# Autodesk Inventor assembly: Frame with winch
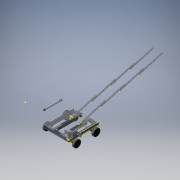
[picture p0: Inventor's stored thumbnail of the model, 180x180]
Saved by Autodesk Inventor 2016 (Build 200138000, 138)
## iProperties
Created: 2015-12-09
Part Number: Frame with winch
Document SubType Name: Assembly
Designer: Julia
Author: Julia
## Documents named in this file (11)
- C:\Users\Julia\Documents\GitHub\RobotuxCAD\FTC CAD Parts\Frame with winch.iam
- C:\Users\Julia\Documents\GitHub\RobotuxCAD\FTC CAD Parts\Frame With Wheels.iam
- C:\Users\Julia\Documents\GitHub\RobotuxCAD\FTC CAD Parts\Tetrix_Kit_FTC\tetrix_739079_collar_2012.ipt
- C:\Users\Julia\Documents\GitHub\RobotuxCAD\FTC CAD Parts\Andy Mark\am-2964NeveRest.ipt
- C:\Users\Julia\Documents\GitHub\RobotuxCAD\FTC CAD Parts\Tetrix_Kit_FTC\tetrix_739089_2012.ipt
- C:\Users\Julia\Documents\GitHub\RobotuxCAD\FTC CAD Parts\Tetrix_Kit_FTC\tetrix_739086_2012.ipt
- C:\Users\Julia\Documents\GitHub\RobotuxCAD\FTC CAD Parts\Tetrix_Kit_FTC\tetrix_739028_2012.ipt
- C:\Users\Julia\Documents\GitHub\RobotuxCAD\FTC CAD Parts\support.ipt
- C:\Users\Julia\Documents\GitHub\RobotuxCAD\FTC CAD Parts\Tetrix_Kit_FTC\tetrix_739172_2012.ipt
- C:\Users\Julia\Documents\GitHub\RobotuxCAD\FTC CAD Parts\tube_clamp_2012.ipt
- C:\Users\Julia\Documents\GitHub\RobotuxCAD\FTC CAD Parts\winch spool.ipt
## Components (13 placed, 10 different names)
1. tetrix_739079_collar_2012:1 — Mate:6, Mate:8, Mate:9
2. am-2964NeveRest:1 — Mate:4, Mate:5, Angle:1, Mate:6, Mate:7
3. tetrix_739089_2012:1 — Mate:1, Mate:2, Mate:3, Mate:4, Mate:5
4. tetrix_739086_2012:1 — Mate:7, Mate:8, Mate:9
5. Frame With Wheels:1 [sub-assembly] — Mate:1, Mate:2, Mate:3, Angle:1, Flush:1, Flush:2, Mate:10, Mate:11
6. tetrix_739028_2012:1 — Mate:12, Mate:13, Mate:14, Mate:15, Mate:16
7. support:1 — Flush:1, Flush:2, Mate:10, Mate:11, Mate:12, Mate:13
8. tetrix_739172_2012:1 — Mate:14, Mate:15, Mate:16
9. tetrix_739172_2012:2 — Mate:17, Mate:19, Mate:22, Mate:23
10. tetrix_739172_2012:3 — Mate:18, Mate:20, Mate:21, Mate:24
11. tube_clamp_2012:1 — Mate:17, Mate:19, Mate:22, Mate:25
12. tube_clamp_2012:2 — Mate:18, Mate:20, Mate:21, Mate:26
13. winch spool:1 — Mate:23, Mate:24, Mate:25, Mate:26
## Relationships (29: Mate 26, Flush 2, Angle 1)
- Mate:1: tetrix_739089_2012:1 ↔ Frame With Wheels:1
- Mate:2: tetrix_739089_2012:1 ↔ Frame With Wheels:1
- Mate:3: tetrix_739089_2012:1 ↔ Frame With Wheels:1
- Mate:4: am-2964NeveRest:1 ↔ tetrix_739089_2012:1
- Mate:5: am-2964NeveRest:1 ↔ tetrix_739089_2012:1
- Angle:1 (0 deg): am-2964NeveRest:1 ↔ Frame With Wheels:1
- Mate:6: tetrix_739079_collar_2012:1 ↔ am-2964NeveRest:1
- Mate:7: am-2964NeveRest:1 ↔ tetrix_739086_2012:1
- Mate:8: tetrix_739079_collar_2012:1 ↔ tetrix_739086_2012:1
- Mate:9: tetrix_739079_collar_2012:1 ↔ tetrix_739086_2012:1
- Flush:1: Frame With Wheels:1 ↔ support:1
- Flush:2: Frame With Wheels:1 ↔ support:1
- Mate:10: Frame With Wheels:1 ↔ support:1
- Mate:11: Frame With Wheels:1 ↔ support:1
- Mate:12: tetrix_739028_2012:1 ↔ support:1
- Mate:13: tetrix_739028_2012:1 ↔ support:1
- Mate:14: tetrix_739028_2012:1 ↔ tetrix_739172_2012:1
- Mate:15: tetrix_739028_2012:1 ↔ tetrix_739172_2012:1
- Mate:16: tetrix_739028_2012:1 ↔ tetrix_739172_2012:1
- Mate:17: tetrix_739172_2012:2 ↔ tube_clamp_2012:1
- Mate:18: tetrix_739172_2012:3 ↔ tube_clamp_2012:2
- Mate:19: tetrix_739172_2012:2 ↔ tube_clamp_2012:1
- Mate:20: tetrix_739172_2012:3 ↔ tube_clamp_2012:2
- Mate:21: tetrix_739172_2012:3 ↔ tube_clamp_2012:2
- Mate:22: tetrix_739172_2012:2 ↔ tube_clamp_2012:1
- Mate:23: tetrix_739172_2012:2 ↔ winch spool:1
- Mate:24: tetrix_739172_2012:3 ↔ winch spool:1
- Mate:25: tube_clamp_2012:1 ↔ winch spool:1
- Mate:26: tube_clamp_2012:2 ↔ winch spool:1
